# Autodesk Inventor assembly: ShedAssembly
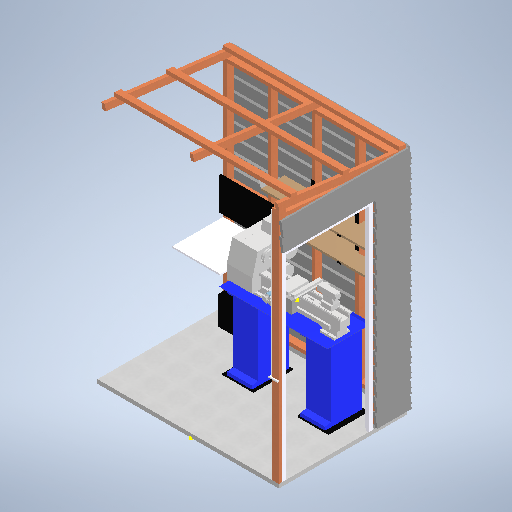
[picture p0: Inventor's stored thumbnail of the model, 512x512]
Saved by Autodesk Inventor 2025.1 (Build 291241000, 241)
## iProperties
Created: 2024-08-20
Part Number: ShedAssembly
Document SubType Name: Assembly
Designer: max_d
Author: max_d
## Documents named in this file (11)
- E:\00 Network Folder\1. Projects\P0. Digital Twins - OTS Parts - Environment Models\Machine Shed\Shed CAD Files\ShedAssembly.iam
- E:\00 Network Folder\1. Projects\P0. Digital Twins - OTS Parts - Environment Models\Machine Shed\Shed CAD Files\MaximaShed.ipt
- E:\00 Network Folder\1. Projects\P0. Digital Twins - OTS Parts - Environment Models\Machine Shed\Shed CAD Files\TopShelf.ipt
- E:\00 Network Folder\1. Projects\P0. Digital Twins - OTS Parts - Environment Models\Machine Shed\Shed CAD Files\BottomShelf.ipt
- E:\00 Network Folder\1. Projects\P0. Digital Twins - OTS Parts - Environment Models\Machine Shed\Shed CAD Files\ShedDesk.ipt
- E:\00 Network Folder\1. Projects\P0. Digital Twins - OTS Parts - Environment Models\Machine Shed\Shed CAD Files\StandLeg.ipt
- E:\00 Network Folder\1. Projects\P0. Digital Twins - OTS Parts - Environment Models\Machine Shed\Shed CAD Files\StandVibrationMat.ipt
- E:\00 Network Folder\1. Projects\P0. Digital Twins - OTS Parts - Environment Models\Machine Shed\Shed CAD Files\ChipTray.ipt
- E:\00 Network Folder\1. Projects\P0. Digital Twins - OTS Parts - Environment Models\Machine Shed\Shed CAD Files\ShedComputer.ipt
- E:\00 Network Folder\1. Projects\P0. Digital Twins - OTS Parts - Environment Models\Machine Shed\Shed CAD Files\ShedMonitor.ipt
- E:\00 Network Folder\1. Projects\P0. Digital Twins - OTS Parts - Environment Models\Machine Shed\Shed CAD Files\AL-250G Lathe Assembly (Stock).iam
## Components (12 placed, 10 different names)
1. MaximaShed:1 — Mate:1, Mate:2, Flush:1, Flush:2, Mate:3, Mate:4, Mate:5, Flush:3, Mate:6, Mate:7, Mate:8, Flush:4, Flush:5, Mate:13, Mate:14, Mate:15, Mate:16, Mate:20
2. TopShelf:1 — Mate:1, Flush:1, Mate:4
3. BottomShelf:1 — Mate:2, Flush:2, Mate:3
4. ShedDesk:1 — Mate:5, Flush:3, Mate:6
5. StandLeg:1 — Mate:10, Mate:12, Mate:16
6. StandLeg:2 — Mate:9, Flush:5, Mate:12, Mate:15, Mate:17, Mate:18, Mate:19
7. StandVibrationMat:1 — Mate:7, Mate:9, Flush:4, Mate:11, Mate:13
8. StandVibrationMat:2 — Mate:8, Mate:10, Mate:11, Mate:14
9. ChipTray:1 — Mate:17, Mate:18, Mate:19, Mate:24, Mate:25, Mate:26
10. ShedComputer:1 — Mate:20
11. ShedMonitor:1
12. AL-250G Lathe Assembly (Stock):1 [sub-assembly] — Mate:24, Mate:25, Mate:26
## Relationships (28: Mate 23, Flush 5)
- Mate:1: MaximaShed:1 ↔ TopShelf:1
- Mate:2: MaximaShed:1 ↔ BottomShelf:1
- Flush:1 (-2.5 mm): MaximaShed:1 ↔ TopShelf:1
- Flush:2 (-2.5 mm): MaximaShed:1 ↔ BottomShelf:1
- Mate:3 (1210 mm): MaximaShed:1 ↔ BottomShelf:1
- Mate:4 (1450 mm): MaximaShed:1 ↔ TopShelf:1
- Mate:5: MaximaShed:1 ↔ ShedDesk:1
- Flush:3: MaximaShed:1 ↔ ShedDesk:1
- Mate:6 (825 mm): MaximaShed:1 ↔ ShedDesk:1
- Mate:7: MaximaShed:1 ↔ StandVibrationMat:1
- Mate:8: MaximaShed:1 ↔ StandVibrationMat:2
- Mate:9: StandLeg:2 ↔ StandVibrationMat:1
- Mate:10: StandLeg:1 ↔ StandVibrationMat:2
- Flush:4 (600 mm): MaximaShed:1 ↔ StandVibrationMat:1
- Mate:11 (440 mm): StandVibrationMat:1 ↔ StandVibrationMat:2
- Flush:5 (645 mm): MaximaShed:1 ↔ StandLeg:2
- Mate:12 (485 mm): StandLeg:1 ↔ StandLeg:2
- Mate:13 (160 mm): MaximaShed:1 ↔ StandVibrationMat:1
- Mate:14 (150 mm): MaximaShed:1 ↔ StandVibrationMat:2
- Mate:15 (175 mm): MaximaShed:1 ↔ StandLeg:2
- Mate:16 (165 mm): MaximaShed:1 ↔ StandLeg:1
- Mate:17: StandLeg:2 ↔ ChipTray:1
- Mate:18 (25 mm): StandLeg:2 ↔ ChipTray:1
- Mate:19 (30 mm): StandLeg:2 ↔ ChipTray:1
- Mate:20: MaximaShed:1 ↔ ShedComputer:1
- Mate:24: ChipTray:1 ↔ AL-250G Lathe Assembly (Stock):1
- Mate:25 (100 mm): ChipTray:1 ↔ AL-250G Lathe Assembly (Stock):1
- Mate:26 (125 mm): ChipTray:1 ↔ AL-250G Lathe Assembly (Stock):1
